# Autodesk Inventor assembly: DriveMotorAssembly
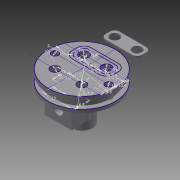
[picture p0: Inventor's stored thumbnail of the model, 180x180]
Saved by Autodesk Inventor 2014 SP1 (Build 180222100, 222)
## iProperties
Created: 2015-03-26
Part Number: DriveMotorAssembly
Document SubType Name: Assembly
Designer: Erin
Author: Erin
## Documents named in this file (3)
- C:\Users\Erin\Desktop\Comp Gen IOAA\DriveMotorAssembly.iam
- C:\Users\Erin\Desktop\Comp Gen IOAA\MotorAttachment.ipt
- C:\Users\Erin\Desktop\Comp Gen IOAA\Winch.ipt
## Components (2 placed, 2 different names)
1. MotorAttachment:1 — Mate:1, Insert:1, Mate:2
2. Winch:1 — Mate:1, Insert:1, Mate:2
## Relationships (3: Mate 2, Insert 1)
- Mate:1: MotorAttachment:1 ↔ Winch:1
- Insert:1: MotorAttachment:1 ↔ Winch:1
- Mate:2: MotorAttachment:1 ↔ Winch:1
